# Autodesk Inventor assembly: scharnier
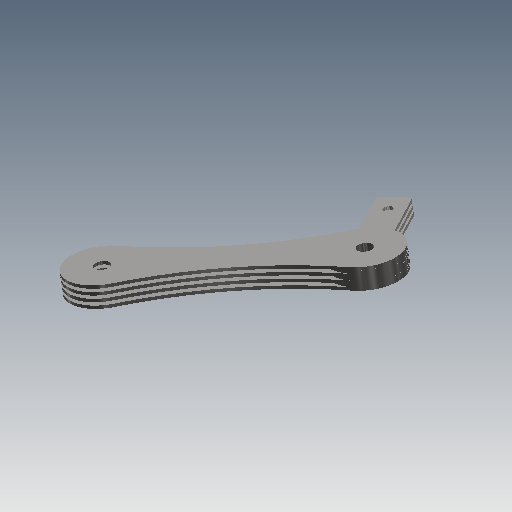
[picture p0: Inventor's stored thumbnail of the model, 512x512]
Saved by Autodesk Inventor 2020.3 (Build 243373000, 373)
## iProperties
Created: 2020-09-15
Part Number: scharnier
Document SubType Name: Assembly
Designer: Svend
Author: Svend
## Documents named in this file (3)
- C:\Users\Svend\OneDrive\Documents\GitHub\Rolstoel\scharnier.iam
- C:\Users\Svend\OneDrive\Documents\GitHub\Rolstoel\stelscharnier bovenkant.ipt
- C:\Users\Svend\OneDrive\Documents\GitHub\Rolstoel\stelscharnier onderkant.ipt
## Components (7 placed, 2 different names)
1. stelscharnier bovenkant:1 — Mate:1, Mate:2, Mate:7, Mate:8, Mate:14, Mate:15
2. stelscharnier onderkant:1 — Mate:1, Mate:2, Mate:9, Mate:10, Mate:12, Mate:16, Mate:17
3. stelscharnier bovenkant:2 — Mate:7, Mate:15
4. stelscharnier onderkant:2 — Mate:8, Mate:16
5. stelscharnier bovenkant:3 — Mate:9, Mate:13, Mate:14
6. stelscharnier onderkant:3 — Mate:10, Mate:11, Mate:17
7. stelscharnier bovenkant:4 — Mate:11, Mate:12, Mate:13
## Relationships (17: Mate 17)
- Mate:1: stelscharnier bovenkant:1 ↔ stelscharnier onderkant:1
- Mate:2: stelscharnier bovenkant:1 ↔ stelscharnier onderkant:1
- [Mate]: stelscharnier bovenkant:2 ↔ stelscharnier onderkant:2
- [Mate]: stelscharnier bovenkant:2 ↔ stelscharnier onderkant:2
- [Mate]: stelscharnier bovenkant:3 ↔ stelscharnier onderkant:3
- [Mate]: stelscharnier bovenkant:3 ↔ stelscharnier onderkant:3
- Mate:7: stelscharnier bovenkant:1 ↔ stelscharnier bovenkant:2
- Mate:8: stelscharnier bovenkant:1 ↔ stelscharnier onderkant:2
- Mate:9: stelscharnier onderkant:1 ↔ stelscharnier bovenkant:3
- Mate:10: stelscharnier onderkant:1 ↔ stelscharnier onderkant:3
- Mate:11: stelscharnier onderkant:3 ↔ stelscharnier bovenkant:4
- Mate:12: stelscharnier onderkant:1 ↔ stelscharnier bovenkant:4
- Mate:13: stelscharnier bovenkant:3 ↔ stelscharnier bovenkant:4
- Mate:14: stelscharnier bovenkant:1 ↔ stelscharnier bovenkant:3
- Mate:15: stelscharnier bovenkant:1 ↔ stelscharnier bovenkant:2
- Mate:16: stelscharnier onderkant:1 ↔ stelscharnier onderkant:2
- Mate:17: stelscharnier onderkant:1 ↔ stelscharnier onderkant:3
## Named parameters: d2_d0 = 0 mm, d3_d1 = 0 mm, d4_d0 = 0 mm, d5_d1 = 0 mm
